# Autodesk Inventor assembly: Thermal Camera Cover Assembly
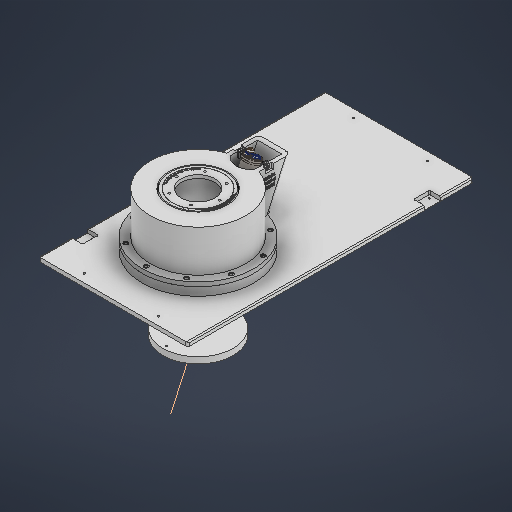
[picture p0: Inventor's stored thumbnail of the model, 512x512]
Saved by Autodesk Inventor 2026.2 (Build 302298000, 298)
## iProperties
Created: 2025-08-06
Part Number: Thermal Camera Cover Assembly
Document SubType Name: Assembly
Designer: mayhe
Author: mayhe
## Documents named in this file (10)
- C:\Users\mayhe\OneDrive\Documents\GitHub\In-situ-monitoring-of-powder-bed-fusion-additive-manufacturing\system_development\Adamant\v0.2\hardware_development\Thermal Camera Cover Assembly.iam
- C:\Users\mayhe\OneDrive\Documents\GitHub\In-situ-monitoring-of-powder-bed-fusion-additive-manufacturing\system_development\Adamant\v0.2\hardware_development\Cover parts\Thermal Chamber Cover.ipt
- C:\Users\mayhe\OneDrive\Documents\GitHub\In-situ-monitoring-of-powder-bed-fusion-additive-manufacturing\system_development\Adamant\v0.2\hardware_development\Cover parts\SealedGlassRing.ipt
- C:\Users\mayhe\OneDrive\Documents\GitHub\In-situ-monitoring-of-powder-bed-fusion-additive-manufacturing\system_development\Adamant\v0.2\hardware_development\Cover parts\Xi-410-Camera-with-29°-x-18°-Lens\Xi 410 Camera with 29° x.iam
- C:\Users\mayhe\OneDrive\Documents\GitHub\In-situ-monitoring-of-powder-bed-fusion-additive-manufacturing\system_development\Adamant\v0.2\hardware_development\Cover parts\substrate plate.ipt
- C:\Users\mayhe\OneDrive\Documents\GitHub\In-situ-monitoring-of-powder-bed-fusion-additive-manufacturing\system_development\Adamant\v0.1\hardware design\Cylinder Segment Holder.ipt
- C:\Users\mayhe\OneDrive\Documents\GitHub\In-situ-monitoring-of-powder-bed-fusion-additive-manufacturing\system_development\Adamant\v0.2\hardware_development\Cover parts\Thermal Housing.ipt
- C:\Users\mayhe\OneDrive\Documents\GitHub\In-situ-monitoring-of-powder-bed-fusion-additive-manufacturing\system_development\Adamant\v0.2\hardware_development\Cover parts\Thermal Cylinder Segments\C .Replace - Face.ipt
- C:\Users\mayhe\OneDrive\Documents\GitHub\In-situ-monitoring-of-powder-bed-fusion-additive-manufacturing\system_development\Adamant\v0.2\hardware_development\Cover parts\Thermal Cylinder Segments.ipt
- C:\Users\mayhe\OneDrive\Documents\GitHub\In-situ-monitoring-of-powder-bed-fusion-additive-manufacturing\system_development\Adamant\v0.2\hardware_development\Cover parts\Thermal Cylinder Segments\C .Replace - 10.ipt
## Components (8 placed, 8 different names)
1. Thermal Chamber Cover:1 — Rotational:1, Mate:1, Rotational:4
2. SealedGlassRing:1 — Rotational:1, Mate:1, Rotational:6
3. Xi 410 Camera with 29° x:1 [sub-assembly] — Rotational:7
4. substrate plate:1 — Rotational:4
5. Cylinder Segment Holder:1
6. Thermal Housing:1 — Rotational:6, Rotational:7, Rotational:8
7. C .Replace - Face:1 — Rotational:8, Rotational:9
8. C .Replace - 10:2 — Rotational:9
## Relationships (7: RevoluteJoint 6, Mate 1)
- Rotational:1 [RevoluteJoint]: Thermal Chamber Cover:1 ↔ SealedGlassRing:1
- Mate:1: Thermal Chamber Cover:1 ↔ SealedGlassRing:1
- Rotational:4 [RevoluteJoint] (-150 mm): Thermal Chamber Cover:1 ↔ substrate plate:1
- Rotational:6 [RevoluteJoint]: SealedGlassRing:1 ↔ Thermal Housing:1
- Rotational:7 [RevoluteJoint]: Xi 410 Camera with 29° x:1 ↔ Thermal Housing:1
- Rotational:8 [RevoluteJoint]: Thermal Housing:1 ↔ C .Replace - Face:1
- Rotational:9 [RevoluteJoint]: C .Replace - Face:1 ↔ C .Replace - 10:2
